# Autodesk Inventor assembly: Budaschnozzle
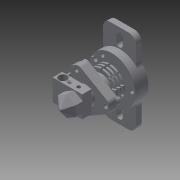
[picture p0: Inventor's stored thumbnail of the model, 180x180]
Saved by Autodesk Inventor 2014 SP1 (Build 180222100, 222)
## iProperties
Created: 2013-12-27
Part Number: Budaschnozzle
Document SubType Name: Assembly
Designer: Jack
Author: Jack
## Documents named in this file (10)
- D:\MendelMax1.5\InventorParts\Hardware\Extruder\Budaschnozzle\Budaschnozzle.iam
- D:\MendelMax1.5\InventorParts\Hardware\Extruder\Budaschnozzle\BackupPlate.ipt
- D:\MendelMax1.5\InventorParts\Hardware\Extruder\Budaschnozzle\Extension.ipt
- D:\MendelMax1.5\InventorParts\Hardware\Extruder\Budaschnozzle\HeaterBlock.ipt
- D:\MendelMax1.5\InventorParts\Hardware\Extruder\Budaschnozzle\HeatSinkWasher.ipt
- D:\MendelMax1.5\InventorParts\Hardware\Extruder\Budaschnozzle\Isolator.ipt
- D:\MendelMax1.5\InventorParts\Hardware\Extruder\Budaschnozzle\LowerPlate.ipt
- D:\MendelMax1.5\InventorParts\Hardware\Extruder\Budaschnozzle\MountPlate.ipt
- D:\MendelMax1.5\InventorParts\Hardware\Extruder\Budaschnozzle\Nozzle.ipt
- D:\MendelMax1.5\InventorParts\Hardware\Extruder\Budaschnozzle\UpperPlate.ipt
## Components (11 placed, 9 different names)
1. BackupPlate:1 — Mate:8, Mate:9, Mate:10, Mate:19
2. Extension:1 — Mate:3, Mate:4, Mate:5
3. HeaterBlock:1 — Mate:1, Mate:2, Mate:3, Mate:6
4. HeatSinkWasher:1 — Mate:11, Mate:12, Mate:13, Mate:14
5. Isolator:1 — Mate:5, Mate:6, Mate:7, Mate:8, Mate:11, Mate:12
6. LowerPlate:1 — Mate:7, Mate:9, Mate:10
7. MountPlate:1 — Mate:20, Mate:21, Mate:22
8. Nozzle:1 — Mate:1, Mate:2, Mate:4
9. UpperPlate:1 — Mate:17, Mate:18, Mate:19, Mate:20, Mate:21, Mate:22
10. HeatSinkWasher:2 — Mate:13, Mate:14, Mate:15, Mate:16
11. HeatSinkWasher:3 — Mate:15, Mate:16, Mate:17, Mate:18
## Relationships (22: Mate 22)
- Mate:1: HeaterBlock:1 ↔ Nozzle:1
- Mate:2: HeaterBlock:1 ↔ Nozzle:1
- Mate:3: Extension:1 ↔ HeaterBlock:1
- Mate:4: Extension:1 ↔ Nozzle:1
- Mate:5: Extension:1 ↔ Isolator:1
- Mate:6: HeaterBlock:1 ↔ Isolator:1
- Mate:7: Isolator:1 ↔ LowerPlate:1
- Mate:8: BackupPlate:1 ↔ Isolator:1
- Mate:9: BackupPlate:1 ↔ LowerPlate:1
- Mate:10: BackupPlate:1 ↔ LowerPlate:1
- Mate:11: HeatSinkWasher:1 ↔ Isolator:1
- Mate:12: HeatSinkWasher:1 ↔ Isolator:1
- Mate:13 (1.5 mm): HeatSinkWasher:1 ↔ HeatSinkWasher:2
- Mate:14: HeatSinkWasher:1 ↔ HeatSinkWasher:2
- Mate:15 (1.5 mm): HeatSinkWasher:2 ↔ HeatSinkWasher:3
- Mate:16: HeatSinkWasher:2 ↔ HeatSinkWasher:3
- Mate:17 (1.5 mm): UpperPlate:1 ↔ HeatSinkWasher:3
- Mate:18: UpperPlate:1 ↔ HeatSinkWasher:3
- Mate:19: BackupPlate:1 ↔ UpperPlate:1
- Mate:20: MountPlate:1 ↔ UpperPlate:1
- Mate:21: MountPlate:1 ↔ UpperPlate:1
- Mate:22: MountPlate:1 ↔ UpperPlate:1
